# Autodesk Inventor assembly: optic
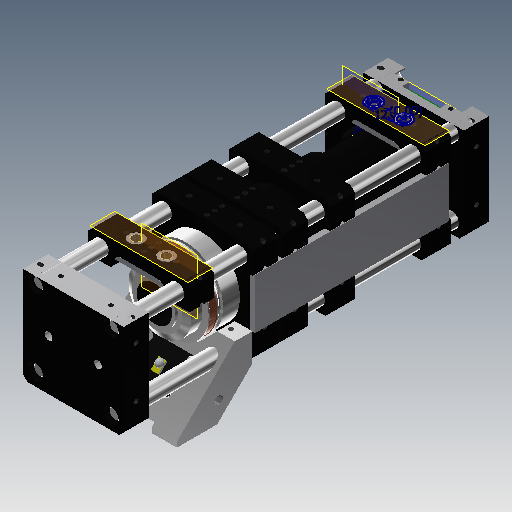
[picture p0: Inventor's stored thumbnail of the model, 512x512]
Saved by Autodesk Inventor 2017 (Build 210142000, 142)
## iProperties
Part Number: optic
Material: Generisch
Document SubType Name: Assembly
Designer: ExCISS
Author: ExCISS
## Documents named in this file (17)
- C:\Seafile\Meine Bibliothek\Inventor\EXCISS\2019\SEU\SEU.iam
- C:\Seafile\Meine Bibliothek\Inventor\EXCISS\2019\SEU\SEU_threaded_insert_M3.ipt
- C:\Seafile\Meine Bibliothek\Inventor\EXCISS\2019\SEU\SEU_threaded_insert_insulation.ipt
- C:\Seafile\Meine Bibliothek\Inventor\EXCISS\2019\SEU\SEU_mounting_fixture_front(G061042000).ipt
- C:\Seafile\Meine Bibliothek\Inventor\EXCISS\2019\SEU\SEU_retaining_plate_HVU.ipt
- C:\Seafile\Meine Bibliothek\Inventor\EXCISS\2019\SEU\SEU_mounting_fixture_back(G061042000).ipt
- C:\Seafile\Meine Bibliothek\Inventor\EXCISS\2019\SEU\SEU_backlight_diffusor_ppma.ipt
- C:\Seafile\Meine Bibliothek\Inventor\EXCISS\2019\SEU\SEU_Luxeon_Rebel_Star_frontlight.ipt
- C:\Seafile\Meine Bibliothek\Inventor\EXCISS\2019\SEU\SEU_led_mount_frontlight.ipt
- C:\Seafile\Meine Bibliothek\Inventor\EXCISS\2019\SEU\SEU_Luxeon_Rebel_Star_backlight.ipt
- C:\Seafile\Meine Bibliothek\Inventor\EXCISS\2019\SEU\SEU_led_mount_backlight_(G061008000).ipt
- C:\Seafile\Meine Bibliothek\Inventor\EXCISS\2019\SEU\SEU_Raspberry_Camera_V2.1.ipt
- C:\Seafile\Meine Bibliothek\Inventor\EXCISS\2019\SEU\SEU_camera_mount_(G061008000).ipt
- C:\Seafile\Meine Bibliothek\Inventor\EXCISS\2019\SEU\SEU_ZEISS_tubus_lense_(423606-8031).ipt
- C:\Seafile\Meine Bibliothek\Inventor\EXCISS\2019\SEU\SEU_LINOS_Microbench_rod_(G061210000).ipt
- C:\Seafile\Meine Bibliothek\Inventor\EXCISS\2019\SEU\SEU_lense_mount_(G061042000).ipt
- C:\Seafile\Meine Bibliothek\Inventor\EXCISS\2019\SEU\SEU_ZEISS_EC_Epiplan-Neofluar_(422320-9900-000).ipt
## Components (26 placed, 16 different names)
1. SEU_ZEISS_EC_Epiplan-Neofluar_(422320-9900-000):1 — Passend:1, Passend:3, Fluchtend:1, Passend:9, Passend:11, Passend:13, Passend:34, Passend:50, Passend:112
2. SEU_lense_mount_(G061042000):1 — Passend:3, Passend:47, Passend:60, Passend:61, Passend:73, Passend:93
3. SEU_LINOS_Microbench_rod_(G061210000):1 — Fluchtend:5, Passend:72, Passend:90
4. SEU_LINOS_Microbench_rod_(G061210000):2 — Fluchtend:4, Fluchtend:5, Fluchtend:6, Fluchtend:12, Passend:60, Passend:62, Passend:63, Passend:64, Passend:66, Passend:77, Passend:89
5. SEU_LINOS_Microbench_rod_(G061210000):3 — Fluchtend:6, Passend:91, Passend:92
6. SEU_LINOS_Microbench_rod_(G061210000):4 — Fluchtend:4, Passend:61, Passend:76, Passend:88, Fluchtend:16
7. SEU_ZEISS_tubus_lense_(423606-8031):1 — Passend:9, Passend:49, Passend:53
8. SEU_lense_mount_(G061042000):2 — Passend:13, Passend:45, Passend:63, Passend:94, Passend:96
9. SEU_lense_mount_(G061042000):3 — Passend:11, Passend:46, Passend:62
10. SEU_camera_mount_(G061008000):1 — Passend:34, Passend:35, Passend:36, Passend:37, Passend:38, Fluchtend:12, Passend:45, Passend:46, Passend:47, Passend:49, Passend:50, Passend:66, Passend:72, Fluchtend:13, Passend:91
11. SEU_Raspberry_Camera_V2.1:1 — Passend:36, Passend:37, Passend:38
12. SEU_led_mount_backlight_(G061008000):1 — Passend:22, Passend:23, Passend:30, Passend:31, Passend:32, Passend:88, Passend:89, Fluchtend:16
13. SEU_Luxeon_Rebel_Star_backlight:1 — Passend:22, Passend:23, Passend:30
14. SEU_led_mount_frontlight:1 — Passend:73, Passend:74, Passend:82, Passend:90, Passend:92, Passend:93, Passend:103
15. SEU_Luxeon_Rebel_Star_frontlight:1 — Passend:74, Passend:82, Passend:103
16. SEU_backlight_diffusor_ppma:1 — Passend:31, Passend:32
17. SEU_mounting_fixture_back(G061042000):1 — Passend:53, Passend:64, Fluchtend:13, Fluchtend:14, Passend:95, Fluchtend:15, Passend:97, Passend:104, Passend:119, Passend:120
18. SEU_retaining_plate_HVU:1 — Passend:94, Fluchtend:14, Passend:95
19. SEU_retaining_plate_HVU:2 — Passend:96, Fluchtend:15, Passend:97
20. SEU_mounting_fixture_front(G061042000):1 — Passend:76, Passend:77, Passend:104, Passend:105, Passend:106, Passend:121
21. SEU_threaded_insert_M3:1 — Passend:102, Passend:107, Passend:109, Passend:110
22. SEU_threaded_insert_M3:2 — Passend:108, Passend:111
23. SEU_threaded_insert_M3:3 — Passend:102, Passend:113, Passend:117, Passend:118
24. SEU_threaded_insert_M3:4 — Passend:114, Passend:115, Passend:116
25. SEU_threaded_insert_insulation:1 — Passend:105, Passend:106, Passend:107, Passend:108, Passend:109, Passend:110, Passend:111, Passend:121
26. SEU_threaded_insert_insulation:2 — Passend:113, Passend:114, Passend:115, Passend:116, Passend:117, Passend:118, Passend:119, Passend:120
## Relationships (72: Mate 63, Flush 9)
- Passend:1 [Mate]: SEU_ZEISS_EC_Epiplan-Neofluar_(422320-9900-000):1
- Passend:3 [Mate]: SEU_ZEISS_EC_Epiplan-Neofluar_(422320-9900-000):1 ↔ SEU_lense_mount_(G061042000):1
- Fluchtend:1 [Flush]: SEU_ZEISS_EC_Epiplan-Neofluar_(422320-9900-000):1
- Fluchtend:4 [Flush]: SEU_LINOS_Microbench_rod_(G061210000):2 ↔ SEU_LINOS_Microbench_rod_(G061210000):4
- Fluchtend:5 [Flush]: SEU_LINOS_Microbench_rod_(G061210000):1 ↔ SEU_LINOS_Microbench_rod_(G061210000):2
- Fluchtend:6 [Flush]: SEU_LINOS_Microbench_rod_(G061210000):2 ↔ SEU_LINOS_Microbench_rod_(G061210000):3
- Passend:9 [Mate]: SEU_ZEISS_EC_Epiplan-Neofluar_(422320-9900-000):1 ↔ SEU_ZEISS_tubus_lense_(423606-8031):1
- Passend:11 [Mate]: SEU_ZEISS_EC_Epiplan-Neofluar_(422320-9900-000):1 ↔ SEU_lense_mount_(G061042000):3
- Passend:13 [Mate]: SEU_ZEISS_EC_Epiplan-Neofluar_(422320-9900-000):1 ↔ SEU_lense_mount_(G061042000):2
- Passend:22 [Mate]: SEU_led_mount_backlight_(G061008000):1 ↔ SEU_Luxeon_Rebel_Star_backlight:1
- Passend:23 [Mate]: SEU_led_mount_backlight_(G061008000):1 ↔ SEU_Luxeon_Rebel_Star_backlight:1
- Passend:30 [Mate]: SEU_led_mount_backlight_(G061008000):1 ↔ SEU_Luxeon_Rebel_Star_backlight:1
- Passend:31 [Mate]: SEU_led_mount_backlight_(G061008000):1 ↔ SEU_backlight_diffusor_ppma:1
- Passend:32 [Mate]: SEU_led_mount_backlight_(G061008000):1 ↔ SEU_backlight_diffusor_ppma:1
- Passend:34 [Mate]: SEU_ZEISS_EC_Epiplan-Neofluar_(422320-9900-000):1 ↔ SEU_camera_mount_(G061008000):1
- Passend:35 [Mate]: SEU_camera_mount_(G061008000):1
- Passend:36 [Mate]: SEU_camera_mount_(G061008000):1 ↔ SEU_Raspberry_Camera_V2.1:1
- Passend:37 [Mate]: SEU_camera_mount_(G061008000):1 ↔ SEU_Raspberry_Camera_V2.1:1
- Passend:38 [Mate]: SEU_camera_mount_(G061008000):1 ↔ SEU_Raspberry_Camera_V2.1:1
- Fluchtend:12 [Flush] (-1.5 mm): SEU_LINOS_Microbench_rod_(G061210000):2 ↔ SEU_camera_mount_(G061008000):1
- Passend:45 [Mate] (43.2 mm): SEU_lense_mount_(G061042000):2 ↔ SEU_camera_mount_(G061008000):1
- Passend:46 [Mate] (61.9 mm): SEU_lense_mount_(G061042000):3 ↔ SEU_camera_mount_(G061008000):1
- Passend:47 [Mate] (73.9 mm): SEU_lense_mount_(G061042000):1 ↔ SEU_camera_mount_(G061008000):1
- Passend:49 [Mate] (9 mm): SEU_ZEISS_tubus_lense_(423606-8031):1 ↔ SEU_camera_mount_(G061008000):1
- Passend:50 [Mate] (-111.8 mm): SEU_ZEISS_EC_Epiplan-Neofluar_(422320-9900-000):1 ↔ SEU_camera_mount_(G061008000):1
- Passend:53 [Mate]: SEU_ZEISS_tubus_lense_(423606-8031):1 ↔ SEU_mounting_fixture_back(G061042000):1
- Passend:60 [Mate]: SEU_lense_mount_(G061042000):1 ↔ SEU_LINOS_Microbench_rod_(G061210000):2
- Passend:61 [Mate]: SEU_lense_mount_(G061042000):1 ↔ SEU_LINOS_Microbench_rod_(G061210000):4
- Passend:62 [Mate]: SEU_LINOS_Microbench_rod_(G061210000):2 ↔ SEU_lense_mount_(G061042000):3
- Passend:63 [Mate]: SEU_LINOS_Microbench_rod_(G061210000):2 ↔ SEU_lense_mount_(G061042000):2
- Passend:64 [Mate]: SEU_LINOS_Microbench_rod_(G061210000):2 ↔ SEU_mounting_fixture_back(G061042000):1
- Passend:66 [Mate]: SEU_LINOS_Microbench_rod_(G061210000):2 ↔ SEU_camera_mount_(G061008000):1
- Passend:72 [Mate]: SEU_LINOS_Microbench_rod_(G061210000):1 ↔ SEU_camera_mount_(G061008000):1
- Passend:73 [Mate]: SEU_lense_mount_(G061042000):1 ↔ SEU_led_mount_frontlight:1
- Passend:74 [Mate]: SEU_led_mount_frontlight:1 ↔ SEU_Luxeon_Rebel_Star_frontlight:1
- Passend:76 [Mate]: SEU_LINOS_Microbench_rod_(G061210000):4 ↔ SEU_mounting_fixture_front(G061042000):1
- Passend:77 [Mate]: SEU_LINOS_Microbench_rod_(G061210000):2 ↔ SEU_mounting_fixture_front(G061042000):1
- Passend:82 [Mate]: SEU_led_mount_frontlight:1 ↔ SEU_Luxeon_Rebel_Star_frontlight:1
- Passend:88 [Mate]: SEU_LINOS_Microbench_rod_(G061210000):4 ↔ SEU_led_mount_backlight_(G061008000):1
- Passend:89 [Mate]: SEU_LINOS_Microbench_rod_(G061210000):2 ↔ SEU_led_mount_backlight_(G061008000):1
- Fluchtend:13 [Flush] (-15 mm): SEU_camera_mount_(G061008000):1 ↔ SEU_mounting_fixture_back(G061042000):1
- Passend:90 [Mate]: SEU_LINOS_Microbench_rod_(G061210000):1 ↔ SEU_led_mount_frontlight:1
- Passend:91 [Mate]: SEU_LINOS_Microbench_rod_(G061210000):3 ↔ SEU_camera_mount_(G061008000):1
- Passend:92 [Mate]: SEU_LINOS_Microbench_rod_(G061210000):3 ↔ SEU_led_mount_frontlight:1
- Passend:93 [Mate]: SEU_lense_mount_(G061042000):1 ↔ SEU_led_mount_frontlight:1
- Passend:94 [Mate]: SEU_lense_mount_(G061042000):2 ↔ SEU_retaining_plate_HVU:1
- Fluchtend:14 [Flush] (-1 mm): SEU_mounting_fixture_back(G061042000):1 ↔ SEU_retaining_plate_HVU:1
- Passend:95 [Mate]: SEU_mounting_fixture_back(G061042000):1 ↔ SEU_retaining_plate_HVU:1
- Passend:96 [Mate]: SEU_lense_mount_(G061042000):2 ↔ SEU_retaining_plate_HVU:2
- Fluchtend:15 [Flush] (1 mm): SEU_mounting_fixture_back(G061042000):1 ↔ SEU_retaining_plate_HVU:2
- Passend:97 [Mate]: SEU_mounting_fixture_back(G061042000):1 ↔ SEU_retaining_plate_HVU:2
- Fluchtend:16 [Flush] (-1.5 mm): SEU_LINOS_Microbench_rod_(G061210000):4 ↔ SEU_led_mount_backlight_(G061008000):1
- Passend:102 [Mate] (-94 mm): SEU_threaded_insert_M3:1 ↔ SEU_threaded_insert_M3:3
- Passend:103 [Mate] (3.8 mm): SEU_led_mount_frontlight:1 ↔ SEU_Luxeon_Rebel_Star_frontlight:1
- Passend:104 [Mate] (84 mm): SEU_mounting_fixture_back(G061042000):1 ↔ SEU_mounting_fixture_front(G061042000):1
- Passend:105 [Mate]: SEU_mounting_fixture_front(G061042000):1 ↔ SEU_threaded_insert_insulation:1
- Passend:106 [Mate]: SEU_mounting_fixture_front(G061042000):1 ↔ SEU_threaded_insert_insulation:1
- Passend:107 [Mate]: SEU_threaded_insert_M3:1 ↔ SEU_threaded_insert_insulation:1
- Passend:108 [Mate]: SEU_threaded_insert_M3:2 ↔ SEU_threaded_insert_insulation:1
- Passend:109 [Mate]: SEU_threaded_insert_M3:1 ↔ SEU_threaded_insert_insulation:1
- Passend:110 [Mate]: SEU_threaded_insert_M3:1 ↔ SEU_threaded_insert_insulation:1
- Passend:111 [Mate]: SEU_threaded_insert_M3:2 ↔ SEU_threaded_insert_insulation:1
- Passend:112 [Mate]: SEU_ZEISS_EC_Epiplan-Neofluar_(422320-9900-000):1
- Passend:113 [Mate]: SEU_threaded_insert_M3:3 ↔ SEU_threaded_insert_insulation:2
- Passend:114 [Mate]: SEU_threaded_insert_M3:4 ↔ SEU_threaded_insert_insulation:2
- Passend:115 [Mate]: SEU_threaded_insert_M3:4 ↔ SEU_threaded_insert_insulation:2
- Passend:116 [Mate]: SEU_threaded_insert_M3:4 ↔ SEU_threaded_insert_insulation:2
- Passend:117 [Mate]: SEU_threaded_insert_M3:3 ↔ SEU_threaded_insert_insulation:2
- Passend:118 [Mate]: SEU_threaded_insert_M3:3 ↔ SEU_threaded_insert_insulation:2
- Passend:119 [Mate]: SEU_mounting_fixture_back(G061042000):1 ↔ SEU_threaded_insert_insulation:2
- Passend:120 [Mate]: SEU_mounting_fixture_back(G061042000):1 ↔ SEU_threaded_insert_insulation:2
- Passend:121 [Mate]: SEU_mounting_fixture_front(G061042000):1 ↔ SEU_threaded_insert_insulation:1
